# Autodesk Inventor assembly: CoreXY Idler 4040 Assembly Left
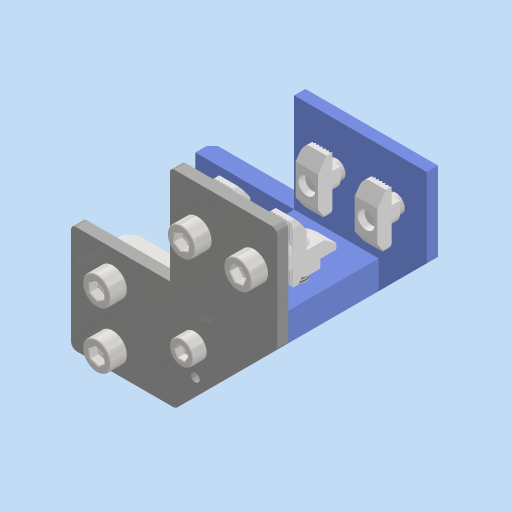
[picture p0: Inventor's stored thumbnail of the model, 512x512]
Saved by Autodesk Inventor 2023.2 (Build 272271000, 271)
## iProperties
Created: 2023-11-27
Part Number: CoreXY Idler 4040 Assembly Left
Document SubType Name: Assembly
Designer: Nils Bade
Author: Nils Bade
## Documents named in this file (13)
- C:\Users\nilsb\Documents\Inventor\Projektarbeit-Bade\RatRig_Bade\CoreXY Idler 4040 Assembly Left.iam
- C:\Users\nilsb\Documents\Inventor\Projektarbeit-Bade\RatRig_modified\xy Idler Left for 4040.ipt
- C:\Users\nilsb\Documents\Inventor\Projektarbeit-Bade\RatRig_modified\Idler Plate for 4040.ipt
- C:\Users\nilsb\Documents\Inventor\Projektarbeit-Bade\Schrauben\Cap Head Screw M5x55 v2.ipt
- C:\Users\nilsb\Documents\Inventor\Projektarbeit-Bade\RatRig_Standards\Hex Locking Nut - M5 v2.ipt
- C:\Users\nilsb\Documents\Inventor\Projektarbeit-Bade\RatRig_modified\T-NUT - DropIn 4040 SERIES - M6.ipt
- C:\Users\nilsb\Documents\Inventor\Projektarbeit-Bade\Schrauben\Cap Head Screw M6x16 - DIN912.ipt
- C:\Users\nilsb\Documents\Inventor\Projektarbeit-Bade\Schrauben\Cap Head Screw M6x12 v2.ipt
- C:\Users\nilsb\Documents\Inventor\Projektarbeit-Bade\Schrauben\Countersink Screw M6x14 v2.ipt
- C:\Users\nilsb\Documents\Inventor\Projektarbeit-Bade\RatRig_Standards\Mini Precision Shim - 8x5x1mm v2.ipt
- C:\Users\nilsb\Documents\Inventor\Projektarbeit-Bade\RatRig_Standards\Ball Bearing - F695ZZ v1.ipt
- C:\Users\nilsb\Documents\Inventor\Projektarbeit-Bade\RatRig_Standards\Ball Bearing - 695ZZ v1.ipt
- C:\Users\nilsb\Documents\Inventor\Projektarbeit-Bade\RatRig_Standards\Aluminium Spacer - 6mm v2.ipt
## Components (28 placed, 12 different names)
1. xy Idler Left for 4040:1 — Fluchtend:2, Fluchtend:3, Passend:1, Passend:5, Winkel:1, Passend:11, Passend:12, Winkel:3, Winkel:8, Passend:15, Passend:18, Passend:19, Winkel:9, Winkel:10, Passend:20, Passend:21, Passend:24, Passend:25, Passend:34, Passend:35, Passend:36, Passend:38, Passend:39, Passend:40
2. Idler Plate for 4040:1 — Fluchtend:2, Fluchtend:3, Passend:1, Passend:2, Passend:3, Passend:6, Passend:7, Passend:8, Passend:9, Winkel:4, Winkel:5, Winkel:6, Winkel:7, Passend:16, Passend:17, Passend:22, Passend:23, Passend:26, Passend:27, Passend:28, Passend:29, Passend:30, Passend:31, Passend:32, Passend:33, Passend:43
3. Cap Head Screw M5x55 v2:1 — Passend:2, Passend:3, Passend:4, Passend:42, Passend:44, Passend:46, Passend:48, Passend:50, Passend:52, Passend:54, Passend:56
4. Hex Locking Nut - M5 v2:1 — Passend:4, Passend:5, Winkel:1
5. T-NUT - DROP IN TYPE FOR 40 SERIES - M6:1 — Winkel:8, Passend:18, Passend:19
6. T-NUT - DROP IN TYPE FOR 40 SERIES - M6:2 — Passend:13, Winkel:10, Passend:21
7. T-NUT - DROP IN TYPE FOR 40 SERIES - M6:3 — Passend:12, Winkel:9, Passend:20
8. T-NUT - DROP IN TYPE FOR 40 SERIES - M6:4 — Passend:11, Winkel:3, Passend:15
9. T-NUT - DROP IN TYPE FOR 40 SERIES - M6:6 — Passend:8, Winkel:5, Passend:17
10. T-NUT - DROP IN TYPE FOR 40 SERIES - M6:7 — Passend:9, Winkel:4, Passend:16
11. T-NUT - DROP IN TYPE FOR 40 SERIES - M6:8 — Passend:6, Winkel:7, Passend:22
12. T-NUT - DROP IN TYPE FOR 40 SERIES - M6:9 — Passend:7, Winkel:6, Passend:23
13. Cap Head Screw M6x16 - DIN912:1 — Passend:24, Passend:25
14. Cap Head Screw M6x12 v2:1 — Passend:29, Passend:33
15. Cap Head Screw M6x12 v2:2 — Passend:28, Passend:32
16. Cap Head Screw M6x12 v2:3 — Passend:26, Passend:30
17. Cap Head Screw M6x12 v2:4 — Passend:27, Passend:31
18. Countersink Screw M6x14 v2:1 — Passend:34, Passend:38, Passend:13
19. Countersink Screw M6x14 v2:2 — Passend:35, Passend:39
20. Countersink Screw M6x14 v2:4 — Passend:36, Passend:40
21. Mini Precision Shim - 8x5x1mm v2:1 — Passend:42, Passend:43, Passend:45
22. Mini Precision Shim - 8x5x1mm v2:2 — Passend:48, Passend:49, Passend:51
23. Mini Precision Shim - 8x5x1mm v2:3 — Passend:56, Passend:57
24. Ball Bearing - F695ZZ v1:1 — Passend:54, Passend:55, Passend:57
25. Ball Bearing - F695ZZ v1:2 — Passend:50, Passend:51, Passend:53
26. Ball Bearing - 695ZZ v1:1 — Passend:52, Passend:53, Passend:55
27. Aluminium Spacer - 6mm v2:1 — Passend:44, Passend:45, Passend:47
28. Aluminium Spacer - 6mm v2:2 — Passend:46, Passend:47, Passend:49
## Relationships (64: Mate 53, Angle 9, Flush 2)
- Fluchtend:2 [Flush]: xy Idler Left for 4040:1 ↔ Idler Plate for 4040:1
- Fluchtend:3 [Flush]: xy Idler Left for 4040:1 ↔ Idler Plate for 4040:1
- Passend:1 [Mate]: xy Idler Left for 4040:1 ↔ Idler Plate for 4040:1
- Passend:2 [Mate]: Idler Plate for 4040:1 ↔ Cap Head Screw M5x55 v2:1
- Passend:3 [Mate]: Idler Plate for 4040:1 ↔ Cap Head Screw M5x55 v2:1
- Passend:4 [Mate]: Cap Head Screw M5x55 v2:1 ↔ Hex Locking Nut - M5 v2:1
- Passend:5 [Mate]: xy Idler Left for 4040:1 ↔ Hex Locking Nut - M5 v2:1
- Winkel:1 [Angle] (0 deg): xy Idler Left for 4040:1 ↔ Hex Locking Nut - M5 v2:1
- Passend:6 [Mate]: Idler Plate for 4040:1 ↔ T-NUT - DROP IN TYPE FOR 40 SERIES - M6:8
- Passend:7 [Mate]: Idler Plate for 4040:1 ↔ T-NUT - DROP IN TYPE FOR 40 SERIES - M6:9
- Passend:8 [Mate]: Idler Plate for 4040:1 ↔ T-NUT - DROP IN TYPE FOR 40 SERIES - M6:6
- Passend:9 [Mate]: Idler Plate for 4040:1 ↔ T-NUT - DROP IN TYPE FOR 40 SERIES - M6:7
- Passend:11 [Mate]: xy Idler Left for 4040:1 ↔ T-NUT - DROP IN TYPE FOR 40 SERIES - M6:4
- Passend:12 [Mate]: xy Idler Left for 4040:1 ↔ T-NUT - DROP IN TYPE FOR 40 SERIES - M6:3
- Passend:13 [Mate]: T-NUT - DROP IN TYPE FOR 40 SERIES - M6:2 ↔ Countersink Screw M6x14 v2:1
- Winkel:3 [Angle] (0 deg): xy Idler Left for 4040:1 ↔ T-NUT - DROP IN TYPE FOR 40 SERIES - M6:4
- Winkel:4 [Angle] (0 deg): Idler Plate for 4040:1 ↔ T-NUT - DROP IN TYPE FOR 40 SERIES - M6:7
- Winkel:5 [Angle] (0 deg): Idler Plate for 4040:1 ↔ T-NUT - DROP IN TYPE FOR 40 SERIES - M6:6
- Winkel:6 [Angle] (0 deg): Idler Plate for 4040:1 ↔ T-NUT - DROP IN TYPE FOR 40 SERIES - M6:9
- Winkel:7 [Angle] (0 deg): Idler Plate for 4040:1 ↔ T-NUT - DROP IN TYPE FOR 40 SERIES - M6:8
- Winkel:8 [Angle] (0 deg): xy Idler Left for 4040:1 ↔ T-NUT - DROP IN TYPE FOR 40 SERIES - M6:1
- Passend:15 [Mate] (5.5 mm): xy Idler Left for 4040:1 ↔ T-NUT - DROP IN TYPE FOR 40 SERIES - M6:4
- Passend:16 [Mate] (5.5 mm): Idler Plate for 4040:1 ↔ T-NUT - DROP IN TYPE FOR 40 SERIES - M6:7
- Passend:17 [Mate] (5.5 mm): Idler Plate for 4040:1 ↔ T-NUT - DROP IN TYPE FOR 40 SERIES - M6:6
- Passend:18 [Mate] (5.5 mm): xy Idler Left for 4040:1 ↔ T-NUT - DROP IN TYPE FOR 40 SERIES - M6:1
- Passend:19 [Mate]: xy Idler Left for 4040:1 ↔ T-NUT - DROP IN TYPE FOR 40 SERIES - M6:1
- Winkel:9 [Angle] (0 deg): xy Idler Left for 4040:1 ↔ T-NUT - DROP IN TYPE FOR 40 SERIES - M6:3
- Winkel:10 [Angle] (0 deg): xy Idler Left for 4040:1 ↔ T-NUT - DROP IN TYPE FOR 40 SERIES - M6:2
- Passend:20 [Mate] (5.5 mm): xy Idler Left for 4040:1 ↔ T-NUT - DROP IN TYPE FOR 40 SERIES - M6:3
- Passend:21 [Mate] (5.5 mm): xy Idler Left for 4040:1 ↔ T-NUT - DROP IN TYPE FOR 40 SERIES - M6:2
- Passend:22 [Mate] (5.5 mm): Idler Plate for 4040:1 ↔ T-NUT - DROP IN TYPE FOR 40 SERIES - M6:8
- Passend:23 [Mate] (5.5 mm): Idler Plate for 4040:1 ↔ T-NUT - DROP IN TYPE FOR 40 SERIES - M6:9
- Passend:24 [Mate]: xy Idler Left for 4040:1 ↔ Cap Head Screw M6x16 - DIN912:1
- Passend:25 [Mate]: xy Idler Left for 4040:1 ↔ Cap Head Screw M6x16 - DIN912:1
- Passend:26 [Mate]: Idler Plate for 4040:1 ↔ Cap Head Screw M6x12 v2:3
- Passend:27 [Mate]: Idler Plate for 4040:1 ↔ Cap Head Screw M6x12 v2:4
- Passend:28 [Mate]: Idler Plate for 4040:1 ↔ Cap Head Screw M6x12 v2:2
- Passend:29 [Mate]: Idler Plate for 4040:1 ↔ Cap Head Screw M6x12 v2:1
- Passend:30 [Mate]: Idler Plate for 4040:1 ↔ Cap Head Screw M6x12 v2:3
- Passend:31 [Mate]: Idler Plate for 4040:1 ↔ Cap Head Screw M6x12 v2:4
- Passend:32 [Mate]: Idler Plate for 4040:1 ↔ Cap Head Screw M6x12 v2:2
- Passend:33 [Mate]: Idler Plate for 4040:1 ↔ Cap Head Screw M6x12 v2:1
- Passend:34 [Mate]: xy Idler Left for 4040:1 ↔ Countersink Screw M6x14 v2:1
- Passend:35 [Mate]: xy Idler Left for 4040:1 ↔ Countersink Screw M6x14 v2:2
- Passend:36 [Mate]: xy Idler Left for 4040:1 ↔ Countersink Screw M6x14 v2:4
- Passend:38 [Mate]: xy Idler Left for 4040:1 ↔ Countersink Screw M6x14 v2:1
- Passend:39 [Mate]: xy Idler Left for 4040:1 ↔ Countersink Screw M6x14 v2:2
- Passend:40 [Mate]: xy Idler Left for 4040:1 ↔ Countersink Screw M6x14 v2:4
- Passend:42 [Mate]: Cap Head Screw M5x55 v2:1 ↔ Mini Precision Shim - 8x5x1mm v2:1
- Passend:43 [Mate]: Idler Plate for 4040:1 ↔ Mini Precision Shim - 8x5x1mm v2:1
- Passend:44 [Mate]: Cap Head Screw M5x55 v2:1 ↔ Aluminium Spacer - 6mm v2:1
- Passend:45 [Mate]: Mini Precision Shim - 8x5x1mm v2:1 ↔ Aluminium Spacer - 6mm v2:1
- Passend:46 [Mate]: Cap Head Screw M5x55 v2:1 ↔ Aluminium Spacer - 6mm v2:2
- Passend:47 [Mate]: Aluminium Spacer - 6mm v2:1 ↔ Aluminium Spacer - 6mm v2:2
- Passend:48 [Mate]: Cap Head Screw M5x55 v2:1 ↔ Mini Precision Shim - 8x5x1mm v2:2
- Passend:49 [Mate]: Mini Precision Shim - 8x5x1mm v2:2 ↔ Aluminium Spacer - 6mm v2:2
- Passend:50 [Mate]: Cap Head Screw M5x55 v2:1 ↔ Ball Bearing - F695ZZ v1:2
- Passend:51 [Mate]: Mini Precision Shim - 8x5x1mm v2:2 ↔ Ball Bearing - F695ZZ v1:2
- Passend:52 [Mate]: Cap Head Screw M5x55 v2:1 ↔ Ball Bearing - 695ZZ v1:1
- Passend:53 [Mate]: Ball Bearing - F695ZZ v1:2 ↔ Ball Bearing - 695ZZ v1:1
- Passend:54 [Mate]: Cap Head Screw M5x55 v2:1 ↔ Ball Bearing - F695ZZ v1:1
- Passend:55 [Mate]: Ball Bearing - F695ZZ v1:1 ↔ Ball Bearing - 695ZZ v1:1
- Passend:56 [Mate]: Cap Head Screw M5x55 v2:1 ↔ Mini Precision Shim - 8x5x1mm v2:3
- Passend:57 [Mate]: Mini Precision Shim - 8x5x1mm v2:3 ↔ Ball Bearing - F695ZZ v1:1
